# Autodesk Inventor assembly: Full Assembly-3
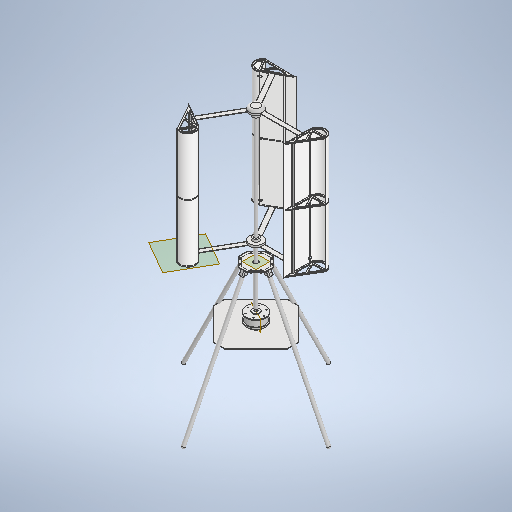
[picture p0: Inventor's stored thumbnail of the model, 512x512]
Saved by Autodesk Inventor 2025.1 (Build 291241000, 241)
## iProperties
Created: 2025-01-29
Part Number: Full Assembly-3
Document SubType Name: Assembly
Designer: Dimas Arif
Author: Dimas Arif
## Documents named in this file (6)
- C:\Users\Dimas Arif\Documents\Inventor\Project-81\Full Assembly-3.iam
- C:\Users\Dimas Arif\Documents\Inventor\Project-81\H1-2.ipt
- C:\Users\Dimas Arif\Documents\Inventor\Project-81\Blade-2.iam
- C:\Users\Dimas Arif\Documents\Inventor\Project-81\Motor.ipt
- C:\Users\Dimas Arif\Documents\Inventor\Content Center Files\R2025\en-US\ISO 4032(2)\ISO 4032 - M8 - ISO.ipt
- C:\Users\Dimas Arif\Documents\Inventor\Content Center Files\R2025\en-US\ISO 4762(2)\ISO 4762 - M8 x 25ISO.ipt
## Components (21 placed, 5 different names)
1. H1-2:1 — Mate:1, Flush:1, Flush:2, Mate:2, Mate:3, Flush:5, Flush:6, Mate:4, Mate:5, Flush:7, Flush:8, Insert:1, Insert:2, Insert:3, Insert:4, Insert:5, Insert:6, Insert:7, Insert:8, Insert:9, Insert:10, Insert:11, Insert:12, Insert:13, Insert:14, Insert:15, Insert:16
2. Blade-2:1 [sub-assembly] — Mate:1, Flush:1, Flush:2, Flush:3, Flush:4
3. Blade-2:2 [sub-assembly] — Mate:2, Flush:4, Flush:5
4. Blade-2:3 [sub-assembly] — Mate:3, Flush:3, Flush:6, Flush:7, Flush:8
5. Motor:1 — Mate:4, Mate:5
6. ISO 4032 M8:1 — Insert:1
7. ISO 4032 M8:2 — Insert:2
8. ISO 4032 M8:3 — Insert:3
9. ISO 4032 M8:4 — Insert:4
10. ISO 4032 M8:5 — Insert:5
11. ISO 4032 M8:6 — Insert:6
12. ISO 4032 M8:7 — Insert:7
13. ISO 4032 M8:8 — Insert:8
14. ISO 4762 M8 x 25:1 — Insert:9
15. ISO 4762 M8 x 25:2 — Insert:10
16. ISO 4762 M8 x 25:3 — Insert:11
17. ISO 4762 M8 x 25:4 — Insert:12
18. ISO 4762 M8 x 25:5 — Insert:13
19. ISO 4762 M8 x 25:6 — Insert:14
20. ISO 4762 M8 x 25:7 — Insert:15
21. ISO 4762 M8 x 25:8 — Insert:16
## Relationships (29: Insert 16, Flush 8, Mate 5)
- Mate:1: H1-2:1 ↔ Blade-2:1
- Flush:1: H1-2:1 ↔ Blade-2:1
- Flush:2 (-60 mm): H1-2:1 ↔ Blade-2:1
- Mate:2: H1-2:1 ↔ Blade-2:2
- Mate:3: H1-2:1 ↔ Blade-2:3
- Flush:3: Blade-2:1 ↔ Blade-2:3
- Flush:4: Blade-2:1 ↔ Blade-2:2
- Flush:5 (-60 mm): H1-2:1 ↔ Blade-2:2
- Flush:6 (-60 mm): H1-2:1 ↔ Blade-2:3
- Mate:4: H1-2:1 ↔ Motor:1
- Mate:5: H1-2:1 ↔ Motor:1
- Flush:7: H1-2:1 ↔ Blade-2:3
- Flush:8: H1-2:1 ↔ Blade-2:3
- Insert:1: H1-2:1 ↔ ISO 4032 M8:1
- Insert:2: H1-2:1 ↔ ISO 4032 M8:2
- Insert:3: H1-2:1 ↔ ISO 4032 M8:3
- Insert:4: H1-2:1 ↔ ISO 4032 M8:4
- Insert:5: H1-2:1 ↔ ISO 4032 M8:5
- Insert:6: H1-2:1 ↔ ISO 4032 M8:6
- Insert:7: H1-2:1 ↔ ISO 4032 M8:7
- Insert:8: H1-2:1 ↔ ISO 4032 M8:8
- Insert:9: H1-2:1 ↔ ISO 4762 M8 x 25:1
- Insert:10: H1-2:1 ↔ ISO 4762 M8 x 25:2
- Insert:11: H1-2:1 ↔ ISO 4762 M8 x 25:3
- Insert:12: H1-2:1 ↔ ISO 4762 M8 x 25:4
- Insert:13: H1-2:1 ↔ ISO 4762 M8 x 25:5
- Insert:14: H1-2:1 ↔ ISO 4762 M8 x 25:6
- Insert:15: H1-2:1 ↔ ISO 4762 M8 x 25:7
- Insert:16: H1-2:1 ↔ ISO 4762 M8 x 25:8
